# Autodesk Inventor assembly: RPiPico
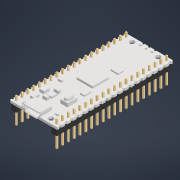
[picture p0: Inventor's stored thumbnail of the model, 180x180]
Saved by Autodesk Inventor 2022 (Build 260153000, 153)
## iProperties
Created: 2021-09-26
Part Number: RPiPico
Document SubType Name: Weldment
Designer: shiok
Weld Material: Welded Aluminum-6061
Author: shiok
## Documents named in this file (3)
- C:\Users\shiok\Documents\GitHub\Keyboard_H\pcb\3D_model\step\RPiPico.iam
- C:\Users\shiok\Documents\GitHub\Keyboard_H\pcb\3D_model\step\PinHeader_1x20_P2.54mm_Vertical.ipt
- C:\Users\shiok\Documents\GitHub\Keyboard_H\pcb\3D_model\step\Pico-R3-step\Pico-R3.iam
## Components (3 placed, 2 different names)
1. PinHeader_1x20_P2.54mm_Vertical:1 — メイト:2
2. PinHeader_1x20_P2.54mm_Vertical:2 — メイト:1
3. Pico-R3:1 [sub-assembly] — メイト:1, メイト:2
## Relationships (2: Mate 2)
- メイト:1 [Mate]: PinHeader_1x20_P2.54mm_Vertical:2 ↔ Pico-R3:1
- メイト:2 [Mate]: PinHeader_1x20_P2.54mm_Vertical:1 ↔ Pico-R3:1
